# Autodesk Inventor assembly: Soporte filamento
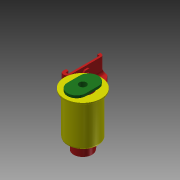
[picture p0: Inventor's stored thumbnail of the model, 180x180]
Saved by Autodesk Inventor 2014 (Build 180170000, 170)
## iProperties
Created: 2017-02-06
Part Number: Soporte filamento
Document SubType Name: Assembly
Designer: Rubén
Author: Rubén
## Documents named in this file (5)
- C:\Users\Rubén\Documents\GitHub\my-3D-printing-designs\Prusa i3 Steel parts\Filament holder\Version #2\Filament holder.iam
- C:\Users\Rubén\Documents\GitHub\my-3D-printing-designs\Prusa i3 Steel parts\Filament holder\Version #2\Filament holder.ipt
- C:\Users\Rubén\Documents\GitHub\my-3D-printing-designs\Prusa i3 Steel parts\Filament holder\Version #2\Adapter for 55mm diameter.ipt
- C:\Users\Rubén\Documents\GitHub\my-3D-printing-designs\Prusa i3 Steel parts\Filament holder\Version #2\Fastener for 70mm width.ipt
- C:\Users\Rubén\Documents\GitHub\my-3D-printing-designs\Prusa i3 Steel parts\Filament holder\Version #2\Fastener for 100mm width.ipt
## Components (4 placed, 4 different names)
1. Filament holder:1 — Mate:1, Flush:1, Mate:2, Angle:1, Mate:3, Mate:4, Mate:5, Angle:2
2. Adapter for 55mm diameter:1 — Mate:1, Flush:1
3. Fastener for 70mm width:1 — Mate:2, Angle:1, Mate:3
4. Fastener for 100mm width:1 — Mate:4, Mate:5, Angle:2
## Relationships (8: Mate 5, Angle 2, Flush 1)
- Mate:1: Filament holder:1 ↔ Adapter for 55mm diameter:1
- Flush:1 (1 mm): Filament holder:1 ↔ Adapter for 55mm diameter:1
- Mate:2: Filament holder:1 ↔ Fastener for 70mm width:1
- Angle:1 (0 deg): Filament holder:1 ↔ Fastener for 70mm width:1
- Mate:3: Filament holder:1 ↔ Fastener for 70mm width:1
- Mate:4: Filament holder:1 ↔ Fastener for 100mm width:1
- Mate:5: Filament holder:1 ↔ Fastener for 100mm width:1
- Angle:2 (0 deg): Filament holder:1 ↔ Fastener for 100mm width:1
